# Autodesk Inventor assembly: FeederV2
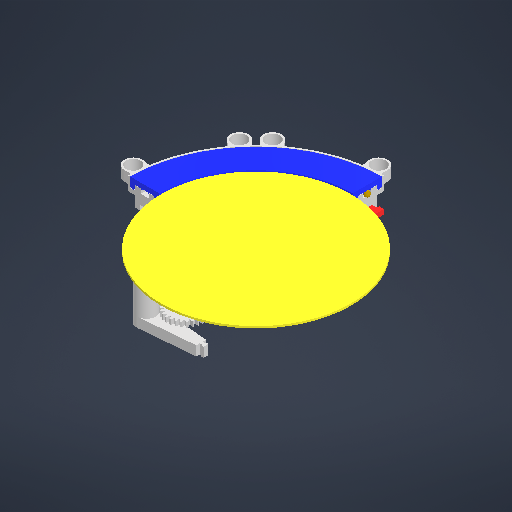
[picture p0: Inventor's stored thumbnail of the model, 512x512]
Saved by Autodesk Inventor 2026 (Build 300175050, 175E)
## iProperties
Created: 2026-03-26
Part Number: FeederV2
Document SubType Name: Assembly
Designer: sniel
Author: sniel
## Documents named in this file (14)
- C:\Users\sniel\OneDrive\SDU\4. Semester\Applied automation\feeder\FeederV2.iam
- C:\Users\sniel\OneDrive\SDU\4. Semester\Applied automation\feeder\base plate.ipt
- C:\Users\sniel\OneDrive\SDU\4. Semester\Applied automation\feeder\outerspinnerV3.ipt
- C:\Users\sniel\OneDrive\SDU\4. Semester\Applied automation\feeder\gears1.ipt
- C:\Users\sniel\OneDrive\SDU\4. Semester\Applied automation\feeder\FeederV2\Design Accelerator\Spur Gears5.iam
- C:\Users\sniel\OneDrive\SDU\4. Semester\Applied automation\feeder\centrer centrifugal spinner.ipt
- C:\Users\sniel\OneDrive\SDU\4. Semester\Applied automation\feeder\central axel.ipt
- C:\Users\sniel\OneDrive\SDU\4. Semester\Applied automation\feeder\base frame.ipt
- C:\Users\sniel\OneDrive\SDU\4. Semester\Applied automation\feeder\moon_gear_V1.ipt
- C:\Users\sniel\OneDrive\SDU\4. Semester\Applied automation\feeder\primlock.ipt
- C:\Users\sniel\OneDrive\SDU\4. Semester\Applied automation\feeder\outerdisk_pin.ipt
- C:\Users\sniel\OneDrive\SDU\4. Semester\Applied automation\feeder\roll_ball_1.ipt
- C:\Users\sniel\OneDrive\SDU\4. Semester\Applied automation\feeder\Leg_v1.ipt
- C:\Users\sniel\OneDrive\SDU\4. Semester\Applied automation\feeder\main axel.ipt
## Components (14 placed, 13 different names)
1. base plate:1
2. outerspinnerV3:1 — Mate:1, Mate:2, Mate:3, Mate:4, Flush:2, Mate:6
3. gears1:1 — Mate:3
4. Spur Gears:4 [sub-assembly] — Mate:1, Mate:2
5. centrer centrifugal spinner:1 — Mate:4, Flush:1
6. central axel:1 — Flush:1, Mate:5, Flush:4
7. base frame:1 — Mate:5, Flush:2, Mate:6, Mate:7, Mate:8, Mate:9, Mate:11, Mate:12, Mate:13, Mate:14
8. moon_gear_V1:1 — Mate:7, Mate:8, Mate:10, Flush:3
9. moon_gear_V1:2 — Mate:9, Mate:11
10. primlock:1 — Mate:10, Flush:3
11. outerdisk_pin:1 — Mate:12
12. roll_ball_1:1
13. Leg_v1:1 — Mate:13, Mate:14
14. main axel:1 — Flush:4
## Relationships (18: Mate 14, Flush 4)
- Mate:1: outerspinnerV3:1 ↔ Spur Gears:4
- Mate:2: outerspinnerV3:1 ↔ Spur Gears:4
- Mate:3: outerspinnerV3:1 ↔ gears1:1
- Mate:4: outerspinnerV3:1 ↔ centrer centrifugal spinner:1
- Flush:1: centrer centrifugal spinner:1 ↔ central axel:1
- Mate:5: central axel:1 ↔ base frame:1
- Flush:2: outerspinnerV3:1 ↔ base frame:1
- Mate:6: outerspinnerV3:1 ↔ base frame:1
- Mate:7: base frame:1 ↔ moon_gear_V1:1
- Mate:8: base frame:1 ↔ moon_gear_V1:1
- Mate:9: base frame:1 ↔ moon_gear_V1:2
- Mate:10: moon_gear_V1:1 ↔ primlock:1
- Flush:3: moon_gear_V1:1 ↔ primlock:1
- Mate:11: base frame:1 ↔ moon_gear_V1:2
- Mate:12: base frame:1 ↔ outerdisk_pin:1
- Mate:13: base frame:1 ↔ Leg_v1:1
- Mate:14: base frame:1 ↔ Leg_v1:1
- Flush:4: central axel:1 ↔ main axel:1
